# Autodesk Inventor assembly: Structure
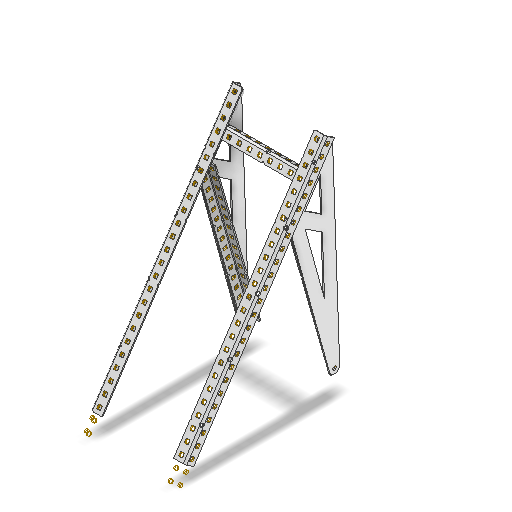
[picture p0: Inventor's stored thumbnail of the model, 512x512]
Saved by Autodesk Inventor 2025.2 (Build 292293000, 293)
## iProperties
Created: 2025-02-15
Part Number: Structure
Document SubType Name: Assembly
Designer: Averey Ku
Author: Averey Ku
## Documents named in this file (6)
- C:\Users\avere\VEX-CAD\V5-CAD\Conveyer\Structure.iam
- C:\Users\avere\VEX-CAD\ROBOPROS-CAD-Inventor\Structure\Angle\Aluminum 1x1\Alu Angle 1x1x16.ipt
- C:\Users\avere\VEX-CAD\V5-CAD\Conveyer\Custom Parts\Triangle Gusset.ipt
- C:\Users\avere\VEX-CAD\ROBOPROS-CAD-Inventor\Motion\Shaft LS\Bearing Flat Low Profile.ipt
- C:\Users\avere\VEX-CAD\ROBOPROS-CAD-Inventor\Structure\Angle\Aluminum 1x1\Alu Angle 1x1x9.ipt
- C:\Users\avere\VEX-CAD\ROBOPROS-CAD-Inventor\Structure\C Channel\Aluminum 1x3x1 Half\Alu C Half 1x3x1x27.ipt
## Components (9 placed, 5 different names)
1. Alu Angle 1x1x16:1 — Mate:7
2. Alu Angle 1x1x16:2 — Mate:8
3. Triangle Gusset:1 — Mate:7
4. Triangle Gusset:2 — Mate:8
5. Bearing Flat Low Profile:1 — Insert:2, Mate:10
6. Bearing Flat Low Profile:2 — Insert:1, Mate:9
7. Alu Angle 1x1x9:1
8. Alu C Half 1x3x1x27:1 — Insert:1, Mate:9
9. Alu C Half 1x3x1x27:2 — Insert:2, Mate:10
## Relationships (7: Mate 5, Insert 2)
- [Mate]: Alu Angle 1x1x16:1 ↔ Triangle Gusset:1
- Mate:7: Alu Angle 1x1x16:1 ↔ Triangle Gusset:1
- Mate:8: Alu Angle 1x1x16:2 ↔ Triangle Gusset:2
- Insert:1 (1.5875 mm): Bearing Flat Low Profile:2 ↔ Alu C Half 1x3x1x27:1
- Mate:9: Bearing Flat Low Profile:2 ↔ Alu C Half 1x3x1x27:1
- Insert:2 (1.5875 mm): Bearing Flat Low Profile:1 ↔ Alu C Half 1x3x1x27:2
- Mate:10: Bearing Flat Low Profile:1 ↔ Alu C Half 1x3x1x27:2
